# Autodesk Inventor assembly: BatteryPack
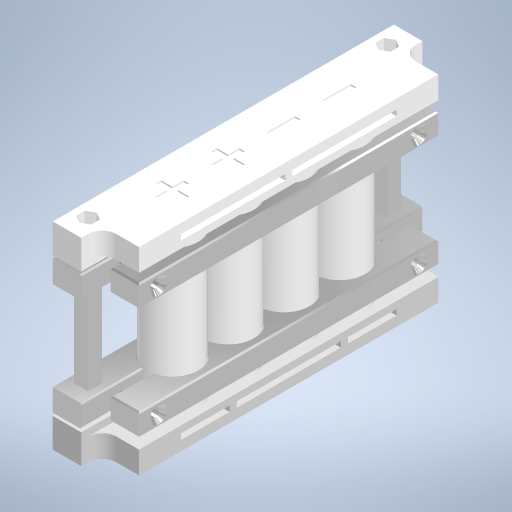
[picture p0: Inventor's stored thumbnail of the model, 512x512]
Saved by Autodesk Inventor 2023 (Build 270158000, 158)
## iProperties
Created: 2022-08-09
Part Number: BatteryPack
Document SubType Name: Assembly
Designer: Aditya Bansal
Author: Aditya Bansal
## Documents named in this file (7)
- C:\Users\Aditya Bansal\OneDrive - UNSW\Uni\BlueSat\rocketry-datasat\Structure\Electronics_Structure\Battery_V1\BatteryPack.iam
- C:\Users\Aditya Bansal\OneDrive - UNSW\Uni\BlueSat\rocketry-datasat\Structure\Electronics_Structure\Battery_V1\BatteryHolderTop.ipt
- C:\Users\Aditya Bansal\OneDrive - UNSW\Uni\BlueSat\rocketry-datasat\Structure\Electronics_Structure\Battery_V1\BatteryHolderBottom.ipt
- C:\Users\Aditya Bansal\OneDrive - UNSW\Uni\BlueSat\rocketry-datasat\Structure\Electronics_Structure\COTS\Battery_Cell_18650.ipt
- C:\Users\Aditya Bansal\OneDrive - UNSW\Uni\BlueSat\rocketry-datasat\Structure\Electronics_Structure\Battery_V1\BatteryStandoff.ipt
- C:\Users\Aditya Bansal\OneDrive - UNSW\Uni\BlueSat\rocketry-datasat\Structure\Electronics_Structure\Battery_V1\BatteryHolderEnd.ipt
- C:\Users\Aditya Bansal\OneDrive - UNSW\Uni\BlueSat\rocketry-datasat\Structure\Electronics_Structure\Battery_V1\BatteryHolderEndSeries.ipt
## Components (12 placed, 6 different names)
1. BatteryHolderBottom:1 — Mate:1, Mate:2, Mate:3, Mate:4, Mate:5, Mate:6, Mate:7, Mate:10, Mate:11, Mate:19, Mate:20, Mate:21, Mate:22, Mate:30
2. BatteryHolderTop:1 — Mate:8, Mate:9, Mate:10, Mate:11
3. Battery_Cell_18650:1 — Mate:4, Flush:2, Mate:8, Mate:17, Mate:24, Mate:27, Mate:28, Mate:29
4. Battery_Cell_18650:2 — Mate:1, Flush:1, Mate:9, Mate:16, Mate:18, Mate:25, Mate:26
5. Battery_Cell_18650:3 — Mate:2, Flush:1, Flush:3
6. Battery_Cell_18650:4 — Mate:3, Flush:2, Flush:3
7. BatteryHolderTop:2 — Mate:18
8. BatteryHolderBottom:2 — Mate:16, Mate:17, Mate:23
9. BatteryStandoff:1 — Mate:19, Mate:22, Mate:23
10. BatteryStandoff:2 — Mate:20, Mate:21
11. BatteryHolderEnd:1 — Mate:26, Mate:27, Mate:29, Mate:30
12. BatteryHolderEndSeries:1 — Mate:24, Mate:25, Mate:28
## Relationships (31: Mate 28, Flush 3)
- Mate:1: BatteryHolderBottom:1 ↔ Battery_Cell_18650:2
- Mate:2: BatteryHolderBottom:1 ↔ Battery_Cell_18650:3
- Mate:3: BatteryHolderBottom:1 ↔ Battery_Cell_18650:4
- Mate:4: BatteryHolderBottom:1 ↔ Battery_Cell_18650:1
- Mate:5: BatteryHolderBottom:1
- Mate:6: BatteryHolderBottom:1
- Mate:7: BatteryHolderBottom:1
- Flush:1: Battery_Cell_18650:2 ↔ Battery_Cell_18650:3
- Flush:2: Battery_Cell_18650:1 ↔ Battery_Cell_18650:4
- Flush:3: Battery_Cell_18650:3 ↔ Battery_Cell_18650:4
- Mate:8: BatteryHolderTop:1 ↔ Battery_Cell_18650:1
- Mate:9: BatteryHolderTop:1 ↔ Battery_Cell_18650:2
- Mate:10: BatteryHolderBottom:1 ↔ BatteryHolderTop:1
- Mate:11: BatteryHolderBottom:1 ↔ BatteryHolderTop:1
- [Mate]: BatteryHolderTop:2 ↔ BatteryHolderBottom:2
- [Mate]: BatteryHolderTop:2 ↔ BatteryHolderBottom:2
- Mate:16: Battery_Cell_18650:2 ↔ BatteryHolderBottom:2
- Mate:17: Battery_Cell_18650:1 ↔ BatteryHolderBottom:2
- Mate:18: Battery_Cell_18650:2 ↔ BatteryHolderTop:2
- Mate:19: BatteryHolderBottom:1 ↔ BatteryStandoff:1
- Mate:20: BatteryHolderBottom:1 ↔ BatteryStandoff:2
- Mate:21: BatteryHolderBottom:1 ↔ BatteryStandoff:2
- Mate:22: BatteryHolderBottom:1 ↔ BatteryStandoff:1
- Mate:23: BatteryHolderBottom:2 ↔ BatteryStandoff:1
- Mate:24: Battery_Cell_18650:1 ↔ BatteryHolderEndSeries:1
- Mate:25: Battery_Cell_18650:2 ↔ BatteryHolderEndSeries:1
- Mate:26: Battery_Cell_18650:2 ↔ BatteryHolderEnd:1
- Mate:27: Battery_Cell_18650:1 ↔ BatteryHolderEnd:1
- Mate:28: Battery_Cell_18650:1 ↔ BatteryHolderEndSeries:1
- Mate:29: Battery_Cell_18650:1 ↔ BatteryHolderEnd:1
- Mate:30 (1 mm): BatteryHolderBottom:1 ↔ BatteryHolderEnd:1
## Named parameters: d15_d14 = 0 mm, d18_d13 = 0 mm
